# Autodesk Inventor assembly: hand
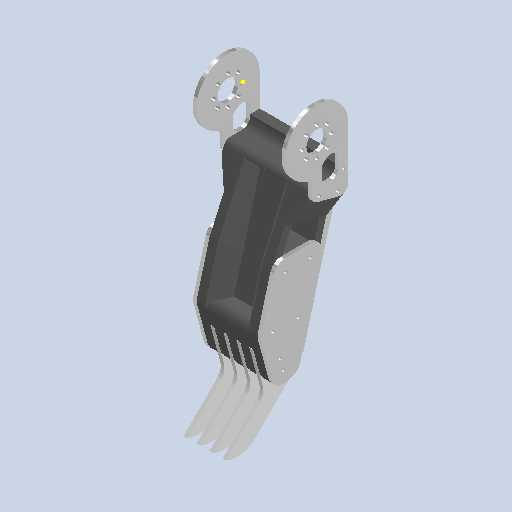
[picture p0: Inventor's stored thumbnail of the model, 512x512]
Saved by Autodesk Inventor 2024.1 (Build 281209000, 209)
## iProperties
Created: 2024-02-14
Part Number: hand
Document SubType Name: Assembly
Designer: hibik
Author: hibik
## Documents named in this file (6)
- C:\Users\hibik\Desktop\ロボメカ\HR\2024.02.11 Rl\02.11 ProtType\hand.iam
- C:\Users\hibik\Desktop\ロボメカ\HR\2024.02.11 Rl\02.11 ProtType\hand_middle.ipt
- C:\Users\hibik\Desktop\ロボメカ\HR\2024.02.11 Rl\02.11 ProtType\elbow_side.ipt
- C:\Users\hibik\Desktop\ロボメカ\HR\2024.02.11 Rl\02.11 ProtType\hand.ipt
- C:\Users\hibik\Desktop\ロボメカ\HR\2024.02.11 Rl\02.11 ProtType\claw2.ipt
- C:\Users\hibik\Desktop\ロボメカ\HR\2024.02.11 Rl\02.11 ProtType\shield.iam
## Components (10 placed, 5 different names)
1. elbow_side:1 — メイト:1, 挿入:1
2. hand_middle:1 — メイト:1, メイト:3, メイト:4, フラッシュ:4, フラッシュ:5, フラッシュ:6, フラッシュ:7, メイト:5, メイト:6, フラッシュ:8, メイト:7, メイト:8, フラッシュ:9, メイト:9, メイト:10, フラッシュ:10, メイト:11, メイト:12, フラッシュ:11, 挿入:1, 挿入:2, 挿入:3, 挿入:4, 挿入:5
3. hand:1 — メイト:4, フラッシュ:4, フラッシュ:7
4. hand:2 — メイト:3, フラッシュ:5, フラッシュ:6
5. claw2:1 — メイト:11, メイト:12, フラッシュ:11
6. claw2:2 — メイト:9, メイト:10, フラッシュ:10
7. claw2:3 — メイト:7, メイト:8, フラッシュ:9
8. claw2:4 — メイト:5, メイト:6, フラッシュ:8
9. elbow_side:2 — 挿入:2, 挿入:3
10. shield:1 [sub-assembly] — 挿入:4, 挿入:5
## Relationships (24: Mate 11, Flush 8, Insert 5)
- メイト:1 [Mate]: elbow_side:1 ↔ hand_middle:1
- メイト:3 [Mate]: hand_middle:1 ↔ hand:2
- メイト:4 [Mate]: hand_middle:1 ↔ hand:1
- フラッシュ:4 [Flush]: hand_middle:1 ↔ hand:1
- フラッシュ:5 [Flush]: hand_middle:1 ↔ hand:2
- フラッシュ:6 [Flush]: hand_middle:1 ↔ hand:2
- フラッシュ:7 [Flush]: hand_middle:1 ↔ hand:1
- メイト:5 [Mate]: hand_middle:1 ↔ claw2:4
- メイト:6 [Mate]: hand_middle:1 ↔ claw2:4
- フラッシュ:8 [Flush]: hand_middle:1 ↔ claw2:4
- メイト:7 [Mate]: hand_middle:1 ↔ claw2:3
- メイト:8 [Mate]: hand_middle:1 ↔ claw2:3
- フラッシュ:9 [Flush]: hand_middle:1 ↔ claw2:3
- メイト:9 [Mate]: hand_middle:1 ↔ claw2:2
- メイト:10 [Mate]: hand_middle:1 ↔ claw2:2
- フラッシュ:10 [Flush]: hand_middle:1 ↔ claw2:2
- メイト:11 [Mate]: hand_middle:1 ↔ claw2:1
- メイト:12 [Mate]: hand_middle:1 ↔ claw2:1
- フラッシュ:11 [Flush]: hand_middle:1 ↔ claw2:1
- 挿入:1 [Insert]: elbow_side:1 ↔ hand_middle:1
- 挿入:2 [Insert]: hand_middle:1 ↔ elbow_side:2
- 挿入:3 [Insert]: hand_middle:1 ↔ elbow_side:2
- 挿入:4 [Insert]: hand_middle:1 ↔ shield:1
- 挿入:5 [Insert]: hand_middle:1 ↔ shield:1
